# Autodesk Inventor assembly: motorAssembly
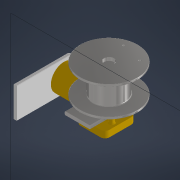
[picture p0: Inventor's stored thumbnail of the model, 180x180]
Saved by Autodesk Inventor 2021 (Build 250183000, 183)
## iProperties
Created: 2021-06-20
Part Number: motorAssembly
Document SubType Name: Assembly
Designer: Watchdog
Author: Watchdog
## Documents named in this file (5)
- C:\Users\Watchdog\OneDrive - Flinders\Advn Mech Design Shared\6_Development\2_Design\inventor\support\reel\motorAssembly.iam
- C:\Users\Watchdog\OneDrive - Flinders\Advn Mech Design Shared\6_Development\2_Design\inventor\support\reel\motor.ipt
- C:\Users\Watchdog\OneDrive - Flinders\Advn Mech Design Shared\6_Development\2_Design\inventor\support\reel\reel.ipt
- C:\Users\Watchdog\OneDrive - Flinders\Advn Mech Design Shared\6_Development\2_Design\inventor\support\reel\motorHolder_stator.ipt
- C:\Users\Watchdog\OneDrive - Flinders\Advn Mech Design Shared\6_Development\2_Design\inventor\support\reel\motorHolder_rotor.ipt
## Components (4 placed, 4 different names)
1. motor:1 — Mate:7, Mate:8, Mate:9, Mate:10, Mate:11, Mate:12, Mate:13, Mate:14
2. reel:1 — Mate:7, Mate:8, Mate:9
3. motorHolder_stator:1 — Mate:10, Mate:11
4. motorHolder_rotor:1 — Mate:12, Mate:13, Mate:14
## Relationships (8: Mate 8)
- Mate:7: motor:1 ↔ reel:1
- Mate:8: motor:1 ↔ reel:1
- Mate:9: motor:1 ↔ reel:1
- Mate:10: motor:1 ↔ motorHolder_stator:1
- Mate:11: motor:1 ↔ motorHolder_stator:1
- Mate:12: motor:1 ↔ motorHolder_rotor:1
- Mate:13: motor:1 ↔ motorHolder_rotor:1
- Mate:14: motor:1 ↔ motorHolder_rotor:1
